# Autodesk Inventor assembly: genelMontaj
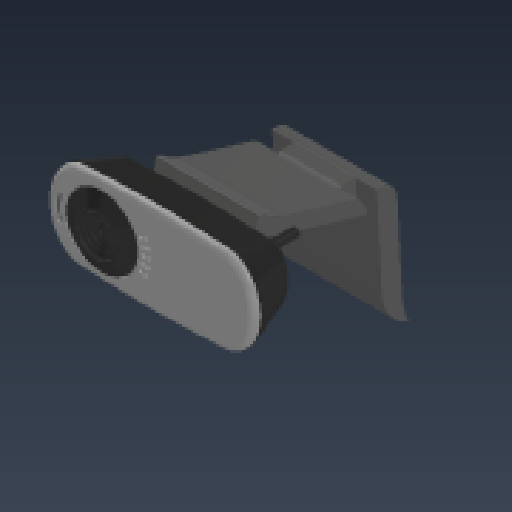
[picture p0: Inventor's stored thumbnail of the model, 512x512]
Saved by Autodesk Inventor 2026 (Build 300175000, 175)
## iProperties
Created: 2021-07-03
Part Number: genelMontaj
Document SubType Name: Assembly
Designer: GameHD
Sending System: SOLIDWORKS 2020
Last Saved Date: 2021-07-03
last saved by: muham
Author: GameHD
## Documents named in this file (4)
- C:\Users\GameHD\Desktop\Phantom 16950\genelMontaj\genelMontaj\genelMontaj.iam
- C:\Users\GameHD\Desktop\Phantom 16950\genelMontaj\genelMontaj\üstKapak.ipt
- C:\Users\GameHD\Desktop\Phantom 16950\genelMontaj\genelMontaj\gövde.ipt
- C:\Users\GameHD\Desktop\Phantom 16950\genelMontaj\genelMontaj\arkaMontaj.iam
## Components (3 placed, 3 different names)
1. üstKapak-1
2. gövde-1 — Совмещение:1
3. arkaMontaj-1 [sub-assembly] — Совмещение:1
## Relationships (1: Mate 1)
- Совмещение:1 [Mate]: gövde-1 ↔ arkaMontaj-1
